# Autodesk Inventor assembly: EMSAMBLAJE_CAMARA_COMBUSTION
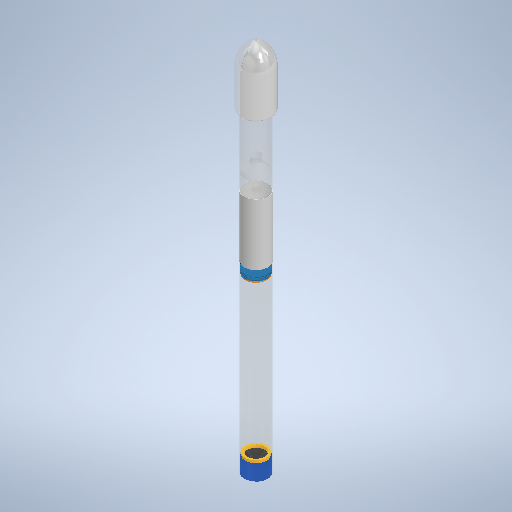
[picture p0: Inventor's stored thumbnail of the model, 512x512]
Saved by Autodesk Inventor 2025 (Build 290162000, 162)
## iProperties
Created: 2024-07-24
Part Number: EMSAMBLAJE_CAMARA_COMBUSTION
Document SubType Name: Assembly
Designer: hansm
Author: hansm
## Documents named in this file (11)
- C:\Users\Richard\3D Objects\ROCKET\EMSAMBLAJE_CAMARA_COMBUSTION.iam
- C:\Users\Richard\3D Objects\ROCKET\CAMARA_DE_COMBUSTION.ipt
- C:\Users\Richard\3D Objects\ROCKET\PARTE_EXTERIOR_TOBERA.ipt
- C:\Users\Richard\3D Objects\ROCKET\PARTE_INTERIOR_FENOLICO_TOBERA.ipt
- C:\Users\Richard\3D Objects\ROCKET\GRAFITO.ipt
- C:\Users\Richard\3D Objects\ROCKET\BASE_INFERIOR_FENOLICO.ipt
- C:\Users\Richard\3D Objects\ROCKET\PARTE_SUPERIOR_IGNICION.ipt
- C:\Users\Richard\3D Objects\ROCKET\BASE_SUPERIOR_FENOLICO.ipt
- C:\Users\Richard\3D Objects\ROCKET\PARACHUTE.ipt
- C:\Users\Richard\3D Objects\ROCKET\ELECTRONIC_PART.ipt
- C:\Users\Richard\3D Objects\ROCKET\PAY-LOAD.ipt
## Components (11 placed, 10 different names)
1. CAMARA_DE_COMBUSTION:1 — Mate:1, Mate:2, Mate:3, Mate:7, Flush:1, Flush:3, Rotational:1
2. PARTE_EXTERIOR_TOBERA:1 — Mate:1, Mate:5, Mate:6, Flush:1, Flush:2
3. PARTE_INTERIOR_FENOLICO_TOBERA:1 — Mate:2, Mate:4, Flush:2
4. GRAFITO:1 — Mate:3, Mate:4
5. BASE_INFERIOR_FENOLICO:1 — Mate:5, Mate:6
6. PARTE_SUPERIOR_IGNICION:1 — Mate:7, Mate:9, Mate:10, Flush:3
7. BASE_SUPERIOR_FENOLICO:1 — Mate:9, Mate:10
8. PARACHUTE:1 — Rotational:2, Rotational:4, Rotational:5
9. ELECTRONIC_PART:1 — Rotational:1, Rotational:2
10. PAY-LOAD:1 — Rotational:5
11. PAY-LOAD:2 — Rotational:4
## Relationships (16: Mate 9, RevoluteJoint 4, Flush 3)
- Mate:1: CAMARA_DE_COMBUSTION:1 ↔ PARTE_EXTERIOR_TOBERA:1
- Mate:2: CAMARA_DE_COMBUSTION:1 ↔ PARTE_INTERIOR_FENOLICO_TOBERA:1
- Mate:3: CAMARA_DE_COMBUSTION:1 ↔ GRAFITO:1
- Mate:4: PARTE_INTERIOR_FENOLICO_TOBERA:1 ↔ GRAFITO:1
- Mate:5: PARTE_EXTERIOR_TOBERA:1 ↔ BASE_INFERIOR_FENOLICO:1
- Mate:6: PARTE_EXTERIOR_TOBERA:1 ↔ BASE_INFERIOR_FENOLICO:1
- Mate:7: CAMARA_DE_COMBUSTION:1 ↔ PARTE_SUPERIOR_IGNICION:1
- Flush:1: CAMARA_DE_COMBUSTION:1 ↔ PARTE_EXTERIOR_TOBERA:1
- Flush:2: PARTE_EXTERIOR_TOBERA:1 ↔ PARTE_INTERIOR_FENOLICO_TOBERA:1
- Mate:9: PARTE_SUPERIOR_IGNICION:1 ↔ BASE_SUPERIOR_FENOLICO:1
- Mate:10: PARTE_SUPERIOR_IGNICION:1 ↔ BASE_SUPERIOR_FENOLICO:1
- Flush:3: CAMARA_DE_COMBUSTION:1 ↔ PARTE_SUPERIOR_IGNICION:1
- Rotational:1 [RevoluteJoint]: CAMARA_DE_COMBUSTION:1 ↔ ELECTRONIC_PART:1
- Rotational:2 [RevoluteJoint]: PARACHUTE:1 ↔ ELECTRONIC_PART:1
- Rotational:4 [RevoluteJoint]: PARACHUTE:1 ↔ PAY-LOAD:2
- Rotational:5 [RevoluteJoint]: PARACHUTE:1 ↔ PAY-LOAD:1
